# Autodesk Inventor assembly: H-Bot_BottomFrame
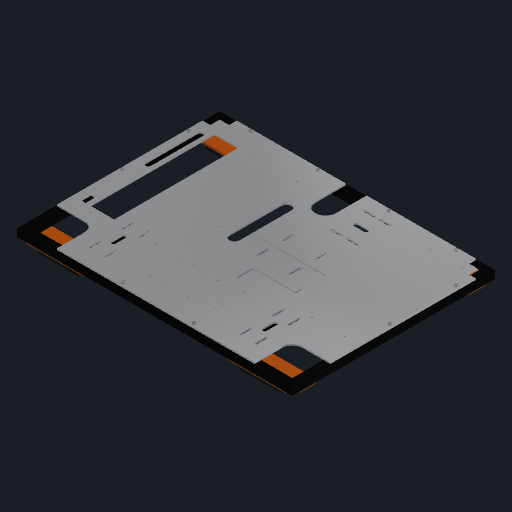
[picture p0: Inventor's stored thumbnail of the model, 512x512]
Saved by Autodesk Inventor 2023.3 (Build 273359000, 359)
## iProperties
Created: 2020-05-24
Part Number: H-Bot_BottomFrame
Document SubType Name: Assembly
Designer: Remo
Description: H-Bot Printer Subassembly / Bottom Frame
Author: Remo
Revision Number: 1.1
## Documents named in this file (9)
- C:\Users\remop\OneDrive\Documents\Inventor\3D Printers\LuEVO\Mk5_FullKinematic\Frame and Panels\Mk5_BottomFrame.iam
- C:\Users\remop\OneDrive\Documents\Inventor\3D Printers\LuEVO\Mk5_FullKinematic\Frame and Panels\Makerbeam\Beam_360mm.ipt
- C:\Users\remop\OneDrive\Documents\Inventor\3D Printers\LuEVO\Mk5_FullKinematic\Frame and Panels\Makerbeam\Beam_CornerCube.ipt
- C:\Users\remop\OneDrive\Documents\Inventor\3D Printers\LuEVO\Mk5_FullKinematic\Frame and Panels\Makerbeam\Beam_CornerTri.ipt
- C:\Users\remop\OneDrive\Documents\Inventor\3D Printers\LuEVO\Mk5_FullKinematic\Frame and Panels\Makerbeam\Beam_500mm.ipt
- C:\Users\remop\OneDrive\Documents\Inventor\3D Printers\LuEVO\Mk5_FullKinematic\Frame and Panels\Makerbeam\Frame_Foot_Solid.ipt
- C:\Users\remop\OneDrive\Documents\Inventor\3D Printers\LuEVO\Mk5_FullKinematic\Frame and Panels\Makerbeam\Frame_Foot_Flex.ipt
- C:\Users\remop\OneDrive\Documents\Inventor\3D Printers\LuEVO\Mk5_FullKinematic\Frame and Panels\BasePlate.ipt
- C:\Users\remop\OneDrive\Documents\Inventor\Content Center Files\R2023\en-US\AS 1420\AS 1420 - 1973 - M3 x 6.ipt
## Components (36 placed, 8 different names)
1. Beam_360mm:1 — Rigid:2, Rigid:3, Mate:2, Mate:27, Mate:28, Flush:22, Mate:35
2. Beam_360mm:2 — Flush:2, Mate:1, Mate:4, Mate:19, Flush:11, Mate:21, Flush:18
3. Beam_360mm:3 — Flush:1, Mate:2, Mate:3, Mate:8, Mate:9, Flush:6, Flush:8
4. Beam_360mm:4 — Rigid:7, Mate:1, Mate:24, Flush:25
5. Beam_CornerCube:1 — Rigid:3, Rigid:4, Flush:15, Flush:29
6. Beam_CornerCube:2 — Rigid:1, Rigid:2, Flush:14, Flush:23
7. Beam_CornerCube:3 — Rigid:6, Flush:19
8. Beam_CornerCube:4 — Rigid:5, Rigid:7, Flush:13, Flush:26
9. Beam_CornerTri:1 — Mate:24, Mate:25, Flush:13
10. Beam_CornerTri:3 — Mate:26, Mate:27, Flush:14
11. Beam_CornerTri:4 — Mate:20, Mate:21, Flush:18
12. Beam_CornerTri:5 — Mate:18, Mate:19, Flush:11
13. Beam_CornerTri:7 — Mate:9, Flush:6, Mate:13
14. Beam_CornerTri:10 — Mate:8, Mate:15, Flush:8
15. Beam_CornerTri:12 — Mate:28, Mate:29, Flush:15
16. Beam_500mm:1 — Rigid:4, Rigid:6, Flush:1, Flush:2, Mate:3, Mate:4, Mate:15, Mate:20, Mate:29, Mate:32, Mate:33, Flush:20, Flush:21, Flush:27
17. Beam_500mm:2 — Rigid:1, Rigid:5, Mate:13, Mate:18, Mate:25, Mate:26, Mate:31, Mate:34, Flush:24
18. BasePlate:1 — Flush:27, Flush:29, Mate:35, Insert:2, Insert:3, Insert:5, Insert:7, Insert:8, Insert:10, Insert:11, Insert:12, Insert:13, Insert:14
19. AS 1420 - Metric M3 x 6:2 — Insert:2
20. AS 1420 - Metric M3 x 6:3 — Insert:3
21. AS 1420 - Metric M3 x 6:5 — Insert:5
22. AS 1420 - Metric M3 x 6:7 — Insert:7
23. AS 1420 - Metric M3 x 6:8 — Insert:8
24. AS 1420 - Metric M3 x 6:10 — Insert:10
25. AS 1420 - Metric M3 x 6:11 — Insert:11
26. AS 1420 - Metric M3 x 6:12 — Insert:12
27. AS 1420 - Metric M3 x 6:13 — Insert:13
28. AS 1420 - Metric M3 x 6:14 — Insert:14
29. Frame_Foot_Solid:1 — Mate:33, Flush:21, Flush:22, Rigid:10
30. Frame_Foot_Solid:2 — Mate:34, Flush:25, Flush:26, Rigid:11
31. Frame_Foot_Solid:3 — Mate:32, Flush:19, Flush:20, Rigid:8
32. Frame_Foot_Solid:4 — Mate:31, Flush:23, Flush:24, Rigid:9
33. Frame_Foot_Flex:1 — Rigid:8
34. Frame_Foot_Flex:2 — Rigid:10
35. Frame_Foot_Flex:3 — Rigid:9
36. Frame_Foot_Flex:4 — Rigid:11
## Relationships (63: Mate 23, Flush 19, WeldJoint 11, Insert 10)
- Rigid:1 [WeldJoint]: Beam_CornerCube:2 ↔ Beam_500mm:2
- Rigid:2 [WeldJoint]: Beam_360mm:1 ↔ Beam_CornerCube:2
- Rigid:3 [WeldJoint]: Beam_360mm:1 ↔ Beam_CornerCube:1
- Rigid:4 [WeldJoint]: Beam_CornerCube:1 ↔ Beam_500mm:1
- Rigid:5 [WeldJoint]: Beam_CornerCube:4 ↔ Beam_500mm:2
- Rigid:6 [WeldJoint]: Beam_CornerCube:3 ↔ Beam_500mm:1
- Rigid:7 [WeldJoint]: Beam_360mm:4 ↔ Beam_CornerCube:4
- Flush:1: Beam_360mm:3 ↔ Beam_500mm:1
- Flush:2: Beam_360mm:2 ↔ Beam_500mm:1
- Mate:1 (100 mm): Beam_360mm:2 ↔ Beam_360mm:4
- Mate:2 (100 mm): Beam_360mm:1 ↔ Beam_360mm:3
- Mate:3: Beam_360mm:3 ↔ Beam_500mm:1
- Mate:4: Beam_360mm:2 ↔ Beam_500mm:1
- Mate:8: Beam_360mm:3 ↔ Beam_CornerTri:10
- Mate:9: Beam_360mm:3 ↔ Beam_CornerTri:7
- Flush:6: Beam_360mm:3 ↔ Beam_CornerTri:7
- Mate:13: Beam_CornerTri:7 ↔ Beam_500mm:2
- Mate:15: Beam_CornerTri:10 ↔ Beam_500mm:1
- Flush:8: Beam_360mm:3 ↔ Beam_CornerTri:10
- Mate:18: Beam_CornerTri:5 ↔ Beam_500mm:2
- Mate:19: Beam_360mm:2 ↔ Beam_CornerTri:5
- Flush:11: Beam_360mm:2 ↔ Beam_CornerTri:5
- Mate:20: Beam_CornerTri:4 ↔ Beam_500mm:1
- Mate:21: Beam_360mm:2 ↔ Beam_CornerTri:4
- Mate:24: Beam_360mm:4 ↔ Beam_CornerTri:1
- Mate:25: Beam_CornerTri:1 ↔ Beam_500mm:2
- Flush:13: Beam_CornerCube:4 ↔ Beam_CornerTri:1
- Mate:26: Beam_CornerTri:3 ↔ Beam_500mm:2
- Mate:27: Beam_360mm:1 ↔ Beam_CornerTri:3
- Flush:14: Beam_CornerCube:2 ↔ Beam_CornerTri:3
- Mate:28: Beam_360mm:1 ↔ Beam_CornerTri:12
- Mate:29: Beam_CornerTri:12 ↔ Beam_500mm:1
- Flush:15: Beam_CornerCube:1 ↔ Beam_CornerTri:12
- Flush:18: Beam_360mm:2 ↔ Beam_CornerTri:4
- Mate:31: Beam_500mm:2 ↔ Frame_Foot_Solid:4
- Mate:32: Beam_500mm:1 ↔ Frame_Foot_Solid:3
- Mate:33: Beam_500mm:1 ↔ Frame_Foot_Solid:1
- Mate:34: Beam_500mm:2 ↔ Frame_Foot_Solid:2
- Flush:19 (2 mm): Beam_CornerCube:3 ↔ Frame_Foot_Solid:3
- Flush:20 (2 mm): Beam_500mm:1 ↔ Frame_Foot_Solid:3
- Flush:21 (-2 mm): Beam_500mm:1 ↔ Frame_Foot_Solid:1
- Flush:22 (2 mm): Beam_360mm:1 ↔ Frame_Foot_Solid:1
- Flush:23 (2 mm): Beam_CornerCube:2 ↔ Frame_Foot_Solid:4
- Flush:24 (-2 mm): Beam_500mm:2 ↔ Frame_Foot_Solid:4
- Flush:25 (2 mm): Beam_360mm:4 ↔ Frame_Foot_Solid:2
- Flush:26 (2 mm): Beam_CornerCube:4 ↔ Frame_Foot_Solid:2
- Rigid:8 [WeldJoint]: Frame_Foot_Solid:3 ↔ Frame_Foot_Flex:1
- Rigid:9 [WeldJoint]: Frame_Foot_Solid:4 ↔ Frame_Foot_Flex:3
- Rigid:10 [WeldJoint]: Frame_Foot_Solid:1 ↔ Frame_Foot_Flex:2
- Rigid:11 [WeldJoint]: Frame_Foot_Solid:2 ↔ Frame_Foot_Flex:4
- Flush:27 (2 mm): Beam_500mm:1 ↔ BasePlate:1
- Flush:29 (2 mm): Beam_CornerCube:1 ↔ BasePlate:1
- Mate:35: Beam_360mm:1 ↔ BasePlate:1
- Insert:2: BasePlate:1 ↔ AS 1420 - Metric M3 x 6:2
- Insert:3: BasePlate:1 ↔ AS 1420 - Metric M3 x 6:3
- Insert:5: BasePlate:1 ↔ AS 1420 - Metric M3 x 6:5
- Insert:7: BasePlate:1 ↔ AS 1420 - Metric M3 x 6:7
- Insert:8: BasePlate:1 ↔ AS 1420 - Metric M3 x 6:8
- Insert:10: BasePlate:1 ↔ AS 1420 - Metric M3 x 6:10
- Insert:11: BasePlate:1 ↔ AS 1420 - Metric M3 x 6:11
- Insert:12: BasePlate:1 ↔ AS 1420 - Metric M3 x 6:12
- Insert:13: BasePlate:1 ↔ AS 1420 - Metric M3 x 6:13
- Insert:14: BasePlate:1 ↔ AS 1420 - Metric M3 x 6:14
